# Autodesk Inventor assembly: motor_core
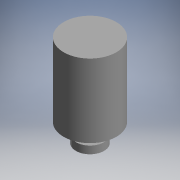
[picture p0: Inventor's stored thumbnail of the model, 180x180]
Saved by Autodesk Inventor 2019.4 (Build 234330000, 330)
## iProperties
Created: 2020-06-20
Part Number: motor_core
Document SubType Name: Assembly
Designer: Jorge
Author: Jorge
## Documents named in this file (4)
- D:\TFG\dev\hardware\ROVER\motor_core.iam
- D:\TFG\dev\hardware\ROVER\motor_body.ipt
- D:\TFG\dev\hardware\ROVER\encoder_pole.ipt
- D:\TFG\dev\hardware\ROVER\encoder_sensor.ipt
## Components (7 placed, 3 different names)
1. motor_body:1 — Mate:1, Flush:1, Mate:2, Flush:2, Mate:4, Flush:3, Mate:6, Flush:4, Flush:5, Mate:8, Mate:9, Mate:10
2. encoder_pole:1 — Mate:1, Flush:1, Mate:3
3. encoder_pole:2 — Mate:2, Mate:3, Flush:2, Mate:5
4. encoder_pole:3 — Mate:4, Mate:5, Flush:3, Mate:7
5. encoder_pole:4 — Mate:6, Mate:7, Flush:4
6. encoder_sensor:1 — Flush:5
7. encoder_sensor:2 — Mate:8, Mate:9, Mate:10
## Relationships (15: Mate 10, Flush 5)
- Mate:1: motor_body:1 ↔ encoder_pole:1
- Flush:1: motor_body:1 ↔ encoder_pole:1
- Mate:2: motor_body:1 ↔ encoder_pole:2
- Mate:3: encoder_pole:1 ↔ encoder_pole:2
- Flush:2: motor_body:1 ↔ encoder_pole:2
- Mate:4: motor_body:1 ↔ encoder_pole:3
- Mate:5: encoder_pole:2 ↔ encoder_pole:3
- Flush:3: motor_body:1 ↔ encoder_pole:3
- Mate:6: motor_body:1 ↔ encoder_pole:4
- Mate:7: encoder_pole:3 ↔ encoder_pole:4
- Flush:4: motor_body:1 ↔ encoder_pole:4
- Flush:5: motor_body:1 ↔ encoder_sensor:1
- Mate:8: motor_body:1 ↔ encoder_sensor:2
- Mate:9: motor_body:1 ↔ encoder_sensor:2
- Mate:10: motor_body:1 ↔ encoder_sensor:2
